# Autodesk Inventor assembly: bett_V2_sitzbank
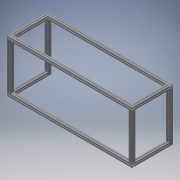
[picture p0: Inventor's stored thumbnail of the model, 180x180]
Saved by Autodesk Inventor 2018 (Build 220112000, 112)
## iProperties
Created: 2020-03-29
Part Number: bett_V2_sitzbank
Material: Generisch
Document SubType Name: Assembly
Designer: wepet
Author: wepet
## Documents named in this file (5)
- C:\Users\wepet\Downloads\anhaenger\current\details\bett\bett_V2_sitzbank.iam
- C:\Users\wepet\Downloads\anhaenger\current\details\bett\details\item_30x30_30cm.ipt
- C:\Users\wepet\Downloads\anhaenger\current\details\bett\details\item_30x30_40cm.ipt
- C:\Users\wepet\Downloads\anhaenger\current\details\bett\details\item_30x30_110cm.ipt
- C:\Users\wepet\Downloads\anhaenger\current\details\bett\details\item_30x30_43cm.ipt
## Components (11 placed, 4 different names)
1. item_30x30_30cm:1 — Fluchtend:2, Passend:3, Fluchtend:3, Fluchtend:31
2. item_30x30_40cm:1 — Fluchtend:4, Passend:4, Fluchtend:5, Passend:6, Fluchtend:15
3. item_30x30_110cm:1 — Passend:1, Passend:2, Fluchtend:1, Fluchtend:2, Passend:3, Fluchtend:3, Fluchtend:4, Passend:4, Fluchtend:5, Fluchtend:8, Fluchtend:9, Fluchtend:10
4. item_30x30_110cm:4 — Fluchtend:8, Fluchtend:9, Passend:6, Fluchtend:11, Fluchtend:16, Passend:8, Fluchtend:23, Fluchtend:25
5. item_30x30_110cm:3 — Fluchtend:10, Fluchtend:11, Fluchtend:24, Fluchtend:26, Fluchtend:27, Fluchtend:28, Fluchtend:30
6. item_30x30_43cm:1 — Fluchtend:29, Fluchtend:30, Fluchtend:31
7. item_30x30_30cm:2 — Fluchtend:15, Fluchtend:16, Passend:8, Fluchtend:29
8. item_30x30_30cm:3 — Fluchtend:20, Fluchtend:22, Passend:12, Fluchtend:32
9. item_30x30_40cm:3 — Fluchtend:19, Fluchtend:21, Passend:12, Fluchtend:25
10. item_30x30_43cm:2 — Fluchtend:18, Fluchtend:21, Passend:9, Passend:10, Fluchtend:28, Fluchtend:32
11. item_30x30_30cm:4 — Fluchtend:18, Fluchtend:19, Fluchtend:20, Fluchtend:22, Passend:9, Passend:10, Fluchtend:23, Fluchtend:24, Fluchtend:26, Fluchtend:27
## Relationships (36: Flush 27, Mate 9)
- Passend:1 [Mate]: item_30x30_110cm:1
- Passend:2 [Mate]: item_30x30_110cm:1
- Fluchtend:1 [Flush]: item_30x30_110cm:1
- Fluchtend:2 [Flush]: item_30x30_30cm:1 ↔ item_30x30_110cm:1
- Passend:3 [Mate]: item_30x30_30cm:1 ↔ item_30x30_110cm:1
- Fluchtend:3 [Flush]: item_30x30_30cm:1 ↔ item_30x30_110cm:1
- Fluchtend:4 [Flush]: item_30x30_40cm:1 ↔ item_30x30_110cm:1
- Passend:4 [Mate]: item_30x30_40cm:1 ↔ item_30x30_110cm:1
- Fluchtend:5 [Flush]: item_30x30_40cm:1 ↔ item_30x30_110cm:1
- Fluchtend:8 [Flush]: item_30x30_110cm:1 ↔ item_30x30_110cm:4
- Fluchtend:9 [Flush]: item_30x30_110cm:1 ↔ item_30x30_110cm:4
- Passend:6 [Mate]: item_30x30_40cm:1 ↔ item_30x30_110cm:4
- Fluchtend:10 [Flush]: item_30x30_110cm:1 ↔ item_30x30_110cm:3
- Fluchtend:11 [Flush]: item_30x30_110cm:4 ↔ item_30x30_110cm:3
- Fluchtend:15 [Flush]: item_30x30_40cm:1 ↔ item_30x30_30cm:2
- Fluchtend:16 [Flush]: item_30x30_110cm:4 ↔ item_30x30_30cm:2
- Passend:8 [Mate]: item_30x30_110cm:4 ↔ item_30x30_30cm:2
- [Flush]: item_30x30_40cm:3 ↔ item_30x30_30cm:4
- Fluchtend:18 [Flush]: item_30x30_43cm:2 ↔ item_30x30_30cm:4
- Fluchtend:19 [Flush]: item_30x30_40cm:3 ↔ item_30x30_30cm:4
- Fluchtend:20 [Flush]: item_30x30_30cm:3 ↔ item_30x30_30cm:4
- Fluchtend:21 [Flush]: item_30x30_40cm:3 ↔ item_30x30_43cm:2
- Fluchtend:22 [Flush]: item_30x30_30cm:3 ↔ item_30x30_30cm:4
- Passend:9 [Mate]: item_30x30_43cm:2 ↔ item_30x30_30cm:4
- Passend:10 [Mate]: item_30x30_43cm:2 ↔ item_30x30_30cm:4
- Passend:12 [Mate]: item_30x30_30cm:3 ↔ item_30x30_40cm:3
- Fluchtend:23 [Flush]: item_30x30_110cm:4 ↔ item_30x30_30cm:4
- Fluchtend:24 [Flush]: item_30x30_110cm:3 ↔ item_30x30_30cm:4
- Fluchtend:25 [Flush]: item_30x30_110cm:4 ↔ item_30x30_40cm:3
- Fluchtend:26 [Flush]: item_30x30_110cm:3 ↔ item_30x30_30cm:4
- Fluchtend:27 [Flush]: item_30x30_110cm:3 ↔ item_30x30_30cm:4
- Fluchtend:28 [Flush]: item_30x30_110cm:3 ↔ item_30x30_43cm:2
- Fluchtend:29 [Flush]: item_30x30_43cm:1 ↔ item_30x30_30cm:2
- Fluchtend:30 [Flush]: item_30x30_110cm:3 ↔ item_30x30_43cm:1
- Fluchtend:31 [Flush]: item_30x30_30cm:1 ↔ item_30x30_43cm:1
- Fluchtend:32 [Flush]: item_30x30_30cm:3 ↔ item_30x30_43cm:2
## Named parameters: d24_d21 = 0 mm
